# Autodesk Inventor assembly: motor assembly (mega troque)
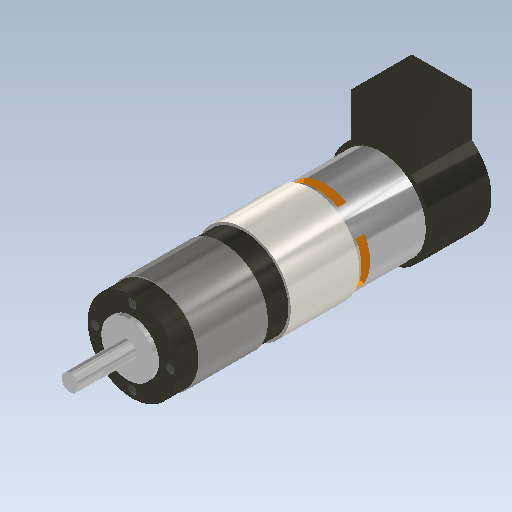
[picture p0: Inventor's stored thumbnail of the model, 512x512]
Saved by Autodesk Inventor 2020 (Build 240168000, 168)
## iProperties
Created: 2020-07-27
Part Number: motor assembly (mega troque)
Document SubType Name: Assembly
Designer: Vikki
Mass: 1751.53 g
Surface Area: 303.485 cm^2
Volume: 223.125 cm^3
Density: 7.85 g/cm^3
Author: Vikki
## Documents named in this file (3)
- E:\project inventor pro\flipkart grid models\articulated arm\motor assembly (mega troque).iam
- E:\project inventor pro\flipkart grid models\articulated arm\motorbody.ipt
- E:\project inventor pro\flipkart grid models\articulated arm\motor_shaft.ipt
## Components (2 placed, 2 different names)
1. motorbody:1 — Mate:1, Mate:2
2. motor_shaft:1 — Mate:1, Mate:2
## Relationships (2: Mate 2)
- Mate:1: motorbody:1 ↔ motor_shaft:1
- Mate:2: motorbody:1 ↔ motor_shaft:1
